# Autodesk Inventor assembly: CHIP_CONTAINER
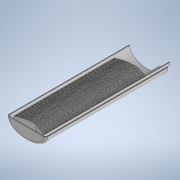
[picture p0: Inventor's stored thumbnail of the model, 180x180]
Saved by Autodesk Inventor 2022 (Build 260153070, 153G)
## iProperties
Created: 2022-04-01
Part Number: CHIP_CONTAINER
Document SubType Name: Assembly
Designer: a laptop
Author: a laptop
## Documents named in this file (4)
- C:\Users\a laptop\Desktop\CADTable_2022_Project\CHIP_CONTAINER.iam
- C:\Users\a laptop\Desktop\CADTable_2022_Project\Container_Design1.ipt
- C:\Users\a laptop\Desktop\CADTable_2022_Project\CHIP.ipt
- C:\Users\a laptop\Desktop\CADTable_2022_Project\chip_holder_V2.ipt
## Components (102 placed, 3 different names)
1. Container_Design1:1 — Mate:3, Angle:2
2. chip_holder_V2:1 — Mate:1, Angle:1, Mate:2, Mate:3, Angle:2
3. CHIP:1 — Mate:1, Angle:1, Mate:2
4. CHIP:2
5. CHIP:3
6. CHIP:4
7. CHIP:5
8. CHIP:6
9. CHIP:7
10. CHIP:8
11. CHIP:9
12. CHIP:10
13. CHIP:11
14. CHIP:12
15. CHIP:13
16. CHIP:14
17. CHIP:15
18. CHIP:16
19. CHIP:17
20. CHIP:18
21. CHIP:19
22. CHIP:20
23. CHIP:21
24. CHIP:22
25. CHIP:23
26. CHIP:24
27. CHIP:25
28. CHIP:26
29. CHIP:27
30. CHIP:28
31. CHIP:29
32. CHIP:30
33. CHIP:31
34. CHIP:32
35. CHIP:33
36. CHIP:34
37. CHIP:35
38. CHIP:36
39. CHIP:37
40. CHIP:38
41. CHIP:39
42. CHIP:40
43. CHIP:41
44. CHIP:42
45. CHIP:43
46. CHIP:44
47. CHIP:45
48. CHIP:46
49. CHIP:47
50. CHIP:48
51. CHIP:49
52. CHIP:50
53. CHIP:51
54. CHIP:52
55. CHIP:53
56. CHIP:54
57. CHIP:55
58. CHIP:56
59. CHIP:57
60. CHIP:58
61. CHIP:59
62. CHIP:60
63. CHIP:61
64. CHIP:62
65. CHIP:63
66. CHIP:64
67. CHIP:65
68. CHIP:66
69. CHIP:67
70. CHIP:68
71. CHIP:69
72. CHIP:70
73. CHIP:71
74. CHIP:72
75. CHIP:73
76. CHIP:74
77. CHIP:75
78. CHIP:76
79. CHIP:77
80. CHIP:78
81. CHIP:79
82. CHIP:80
83. CHIP:81
84. CHIP:82
85. CHIP:83
86. CHIP:84
87. CHIP:85
88. CHIP:86
89. CHIP:87
90. CHIP:88
91. CHIP:89
92. CHIP:90
93. CHIP:91
94. CHIP:92
95. CHIP:93
96. CHIP:94
97. CHIP:95
98. CHIP:96
99. CHIP:97
100. CHIP:98
101. CHIP:99
102. CHIP:100
## Component patterns: (100 elements, first: CHIP:1)
## Relationships (5: Mate 3, Angle 2)
- Mate:1: chip_holder_V2:1 ↔ CHIP:1
- Angle:1 (0 deg): chip_holder_V2:1 ↔ CHIP:1
- Mate:2: chip_holder_V2:1 ↔ CHIP:1
- Mate:3: Container_Design1:1 ↔ chip_holder_V2:1
- Angle:2 (0 deg): Container_Design1:1 ↔ chip_holder_V2:1
